# Autodesk Inventor assembly: Electromagnet final_key
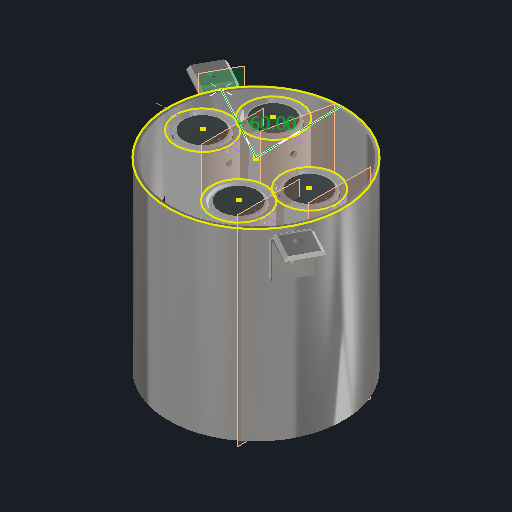
[picture p0: Inventor's stored thumbnail of the model, 512x512]
Saved by Autodesk Inventor 2026.3 (Build 303398000, 398)
## iProperties
Created: 2026-08-03
Part Number: Electromagnet final_key
Document SubType Name: Weldment
Designer: matot
Weld Material: Welded Aluminum-6061
Author: matot
## Documents named in this file (5)
- C:\Users\matot\OneDrive - Stellenbosch University\2026\MechatronicsProject478\Building the joint\Joint Assembly\Electromagnet final_key.iam
- C:\Users\matot\OneDrive - Stellenbosch University\2026\MechatronicsProject478\Building the joint\Joint Assembly\Solenoid Yoke.ipt
- C:\Users\matot\OneDrive - Stellenbosch University\2026\MechatronicsProject478\Building the joint\Joint Assembly\Solenoid core.ipt
- C:\Users\matot\OneDrive - Stellenbosch University\2026\MechatronicsProject478\Building the joint\Joint Assembly\Electromagnet cover_po.iam
- C:\Users\matot\OneDrive - Stellenbosch University\2026\MechatronicsProject478\Building the joint\Joint Assembly\Pressure plate tab_L.ipt
## Components (11 placed, 4 different names)
1. Solenoid Yoke:1 — Insert:1, Insert:9
2. Solenoid core:1 — Insert:1
3. Solenoid Yoke:2 — Insert:2, Insert:8
4. Solenoid core:2 — Insert:2
5. Solenoid Yoke:3 — Insert:4, Insert:7
6. Solenoid core:3 — Insert:4
7. Solenoid Yoke:4 — Insert:3, Insert:6
8. Solenoid core:4 — Insert:3
9. Electromagnet cover_po:1 [sub-assembly] — Insert:6, Insert:7, Insert:8, Insert:9, Tangent:2, Mate:1, Flush:1, Tangent:3, Mate:2, Flush:2
10. Pressure plate tab_L:4 — Tangent:2, Mate:1, Flush:1
11. Pressure plate tab_L:5 — Tangent:3, Mate:2, Flush:2
## Relationships (14: Insert 8, Tangent 2, Mate 2, Flush 2)
- Insert:1: Solenoid Yoke:1 ↔ Solenoid core:1
- Insert:2: Solenoid Yoke:2 ↔ Solenoid core:2
- Insert:3: Solenoid Yoke:4 ↔ Solenoid core:4
- Insert:4: Solenoid Yoke:3 ↔ Solenoid core:3
- Insert:6 (-110 mm): Solenoid Yoke:4 ↔ Electromagnet cover_po:1
- Insert:7 (110 mm): Solenoid Yoke:3 ↔ Electromagnet cover_po:1
- Insert:8 (-110 mm): Solenoid Yoke:2 ↔ Electromagnet cover_po:1
- Insert:9 (110 mm): Solenoid Yoke:1 ↔ Electromagnet cover_po:1
- Tangent:2: Electromagnet cover_po:1 ↔ Pressure plate tab_L:4
- Mate:1: Electromagnet cover_po:1 ↔ Pressure plate tab_L:4
- Flush:1: Electromagnet cover_po:1 ↔ Pressure plate tab_L:4
- Tangent:3: Electromagnet cover_po:1 ↔ Pressure plate tab_L:5
- Mate:2: Electromagnet cover_po:1 ↔ Pressure plate tab_L:5
- Flush:2: Electromagnet cover_po:1 ↔ Pressure plate tab_L:5
